# Autodesk Inventor assembly: FINGER_asm
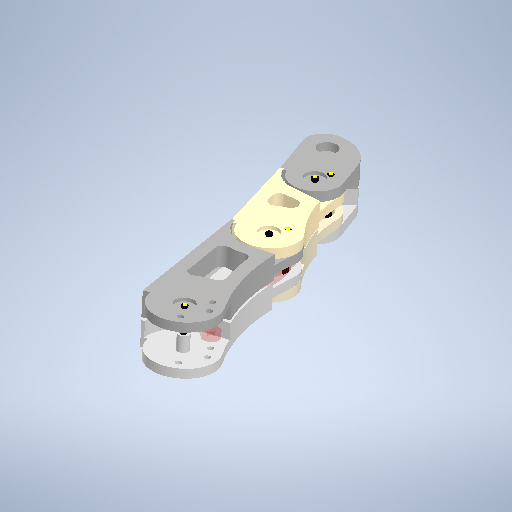
[picture p0: Inventor's stored thumbnail of the model, 512x512]
Saved by Autodesk Inventor 2025.2 (Build 292293000, 293)
## iProperties
Created: 2024-11-09
Part Number: FINGER_asm
Document SubType Name: Assembly
Designer: esandor
Author: esandor
## Documents named in this file (11)
- C:\Users\esandor\Documents\Inventor\INDACT_EE\again\FINGER\FINGER_asm.iam
- C:\Users\esandor\Documents\Inventor\INDACT_EE\again\FINGER\FIN_phalanx_distal_base.ipt
- C:\Users\esandor\Documents\Inventor\INDACT_EE\again\FINGER\FIN_phalanx_media_base.ipt
- C:\Users\esandor\Documents\Inventor\INDACT_EE\again\FINGER\FIN_phalanx_proximal_base.ipt
- C:\Users\esandor\Documents\Inventor\INDACT_EE\again\FINGER\FIN_phalanx_distal_top.ipt
- C:\Users\esandor\Documents\Inventor\INDACT_EE\again\FINGER\FIN_phalanx_media_top.ipt
- C:\Users\esandor\Documents\Inventor\INDACT_EE\again\FINGER\FIN_dowel_pin_long.ipt
- C:\Users\esandor\Documents\Inventor\INDACT_EE\again\FINGER\FIN_phalanx_proximal_top.ipt
- C:\Users\esandor\Documents\Inventor\INDACT_EE\again\FINGER\FIN_dowel_pin_short.ipt
- C:\Users\esandor\Documents\Inventor\INDACT_EE\again\FINGER\FIN_mech_distal.ipt
- C:\Users\esandor\Documents\Inventor\INDACT_EE\again\FINGER\FIN_mech_proximal.ipt
## Components (15 placed, 10 different names)
1. FIN_phalanx_distal_base:1 — Mate:1, Rotational:1, Mate:3, Insert:1, Insert:2, Insert:5, Insert:9
2. FIN_phalanx_media_base:1 — Mate:1, Rotational:1, Insert:4, Rotational:2, Insert:10
3. FIN_phalanx_distal_top:1 — Mate:3, Insert:1, Insert:2, Mate:4, Insert:3, Tangent:3
4. FIN_phalanx_media_top:1 — Mate:4, Insert:3, Tangent:1, Insert:6
5. FIN_dowel_pin_long:1 — Insert:4, Tangent:1
6. FIN_dowel_pin_long:2 — Insert:5, Insert:8
7. FIN_phalanx_proximal_base:1 — Rotational:2, Insert:7, Insert:11, Insert:12
8. FIN_phalanx_proximal_top:1 — Insert:6, Tangent:2, Mate:6, Tangent:6
9. FIN_dowel_pin_long:3 — Insert:7, Tangent:2
10. FIN_dowel_pin_long:4 — Insert:8
11. FIN_dowel_pin_long:6 — Insert:9, Tangent:3, Tangent:4
12. FIN_dowel_pin_long:7 — Insert:10, Tangent:5
13. FIN_dowel_pin_short:1 — Insert:11
14. FIN_mech_distal:1 — Insert:12, Tangent:4
15. FIN_mech_proximal:1 — Tangent:5, Mate:6, Tangent:6
## Relationships (24: Insert 12, Tangent 6, Mate 4, RevoluteJoint 2)
- Mate:1: FIN_phalanx_distal_base:1 ↔ FIN_phalanx_media_base:1
- Rotational:1 [RevoluteJoint]: FIN_phalanx_distal_base:1 ↔ FIN_phalanx_media_base:1
- Mate:3: FIN_phalanx_distal_base:1 ↔ FIN_phalanx_distal_top:1
- Insert:1: FIN_phalanx_distal_base:1 ↔ FIN_phalanx_distal_top:1
- Insert:2: FIN_phalanx_distal_base:1 ↔ FIN_phalanx_distal_top:1
- Mate:4: FIN_phalanx_distal_top:1 ↔ FIN_phalanx_media_top:1
- Insert:3: FIN_phalanx_distal_top:1 ↔ FIN_phalanx_media_top:1
- Insert:4 (-0.8 mm): FIN_phalanx_media_base:1 ↔ FIN_dowel_pin_long:1
- Tangent:1: FIN_phalanx_media_top:1 ↔ FIN_dowel_pin_long:1
- Insert:5 (-1 mm): FIN_phalanx_distal_base:1 ↔ FIN_dowel_pin_long:2
- Rotational:2 [RevoluteJoint]: FIN_phalanx_media_base:1 ↔ FIN_phalanx_proximal_base:1
- Insert:6: FIN_phalanx_media_top:1 ↔ FIN_phalanx_proximal_top:1
- Insert:7 (-0.6 mm): FIN_phalanx_proximal_base:1 ↔ FIN_dowel_pin_long:3
- Tangent:2: FIN_phalanx_proximal_top:1 ↔ FIN_dowel_pin_long:3
- Insert:8: FIN_dowel_pin_long:2 ↔ FIN_dowel_pin_long:4
- Insert:9: FIN_phalanx_distal_base:1 ↔ FIN_dowel_pin_long:6
- Tangent:3: FIN_phalanx_distal_top:1 ↔ FIN_dowel_pin_long:6
- Insert:10 (0.2 mm): FIN_phalanx_media_base:1 ↔ FIN_dowel_pin_long:7
- Insert:11: FIN_phalanx_proximal_base:1 ↔ FIN_dowel_pin_short:1
- Insert:12: FIN_phalanx_proximal_base:1 ↔ FIN_mech_distal:1
- Tangent:4: FIN_dowel_pin_long:6 ↔ FIN_mech_distal:1
- Tangent:5: FIN_dowel_pin_long:7 ↔ FIN_mech_proximal:1
- Mate:6: FIN_phalanx_proximal_top:1 ↔ FIN_mech_proximal:1
- Tangent:6: FIN_phalanx_proximal_top:1 ↔ FIN_mech_proximal:1
